# Autodesk Inventor assembly: Leg_joint_roll_pitch
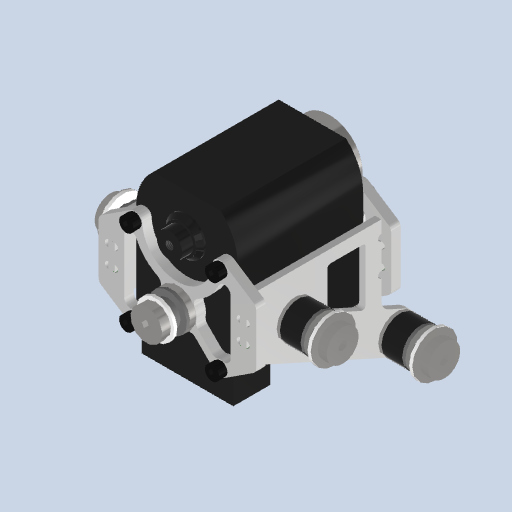
[picture p0: Inventor's stored thumbnail of the model, 512x512]
Saved by Autodesk Inventor 2022 (Build 260153000, 153)
## iProperties
Created: 2022-06-15
Part Number: Leg_joint_roll_pitch
Document SubType Name: Assembly
Designer: Masato Kubotera
Author: Masato Kubotera
## Documents named in this file (21)
- C:\Users\MasatoKubotera\Desktop\SUSTAINA-OP\LowerBody\Leg_joint\Leg_joint_roll_pitch.iam
- C:\Users\MasatoKubotera\Desktop\SUSTAINA-OP\LowerBody\Leg_joint\Leg_joint_pitch_frame.ipt
- C:\Users\MasatoKubotera\Desktop\SUSTAINA-OP\LowerBody\Leg_joint\Leg_joint_roll_frame.ipt
- C:\Users\MasatoKubotera\Desktop\SUSTAINA-OP\ReadyMade\KONDO\B3M-SC-1170-A_with_ClampHorn.iam
- C:\Users\MasatoKubotera\Desktop\SUSTAINA-OP\ReadyMade\InsertNut\S4-05-3W.ipt
- C:\Users\MasatoKubotera\Desktop\SUSTAINA-OP\ReadyMade\InsertNut\SF419.ipt
- C:\Users\MasatoKubotera\Desktop\SUSTAINA-OP\ReadyMade\Spacer\SLSBF6-39.5-M4-N4.ipt
- C:\Users\MasatoKubotera\Desktop\SUSTAINA-OP\ReadyMade\Washer\UUW-0412-10H.ipt
- C:\Users\MasatoKubotera\Desktop\SUSTAINA-OP\ReadyMade\Washer\CCC-0612-65B.ipt
- C:\Users\MasatoKubotera\Desktop\SUSTAINA-OP\ReadyMade\Bush\80F-0603.ipt
- C:\Users\MasatoKubotera\Desktop\SUSTAINA-OP\ReadyMade\Screw\DBTS4-11-6-DHC.ipt
- C:\Users\MasatoKubotera\Desktop\SUSTAINA-OP\ReadyMade\Screw\DBTS4-11-8-DHC.ipt
- C:\Users\MasatoKubotera\Desktop\SUSTAINA-OP\ReadyMade\Screw\DBTS4-5-5-DHC.ipt
- C:\Users\MasatoKubotera\Desktop\SUSTAINA-OP\ReadyMade\Screw\DBTS4-10-4-DHC.ipt
- C:\Users\MasatoKubotera\Desktop\SUSTAINA-OP\ReadyMade\Washer\UUW-0412-20H.ipt
- C:\Users\MasatoKubotera\Desktop\SUSTAINA-OP\ReadyMade\Washer\CC-0612-50B.ipt
- C:\Users\MasatoKubotera\Desktop\SUSTAINA-OP\ReadyMade\Washer\TT-0612-10.ipt
- C:\Users\MasatoKubotera\Desktop\SUSTAINA-OP\ReadyMade\Washer\TT-0814-10.ipt
- C:\Users\MasatoKubotera\Desktop\SUSTAINA-OP\ReadyMade\Washer\UUW-0614-03H.ipt
- C:\Users\MasatoKubotera\Desktop\SUSTAINA-OP\ReadyMade\Screw\FC-2620EB.ipt
- C:\Users\MasatoKubotera\Desktop\SUSTAINA-OP\ReadyMade\Screw\FC-2615EB.ipt
## Components (49 placed, 20 different names)
1. Leg_joint_pitch_frame:1 — 挿入:1, メイト:3, メイト:4, フラッシュ:2, フラッシュ:3, 挿入:13, 挿入:15, 挿入:16
2. Leg_joint_roll_frame:1 — 挿入:3, 角度:1, 挿入:5, 挿入:6, 挿入:7, 挿入:8, メイト:3, メイト:4, フラッシュ:2, メイト:5, メイト:6, 挿入:31, 挿入:48, 挿入:49, 挿入:50, 挿入:51
3. Leg_joint_pitch_frame:2 — 挿入:2, メイト:5, メイト:6, フラッシュ:3, 挿入:14, 挿入:17, 挿入:18
4. Leg_joint_roll_frame:2 — 挿入:4, 角度:2, 挿入:9, 挿入:10, 挿入:11, 挿入:12, 挿入:32, 挿入:52, 挿入:53
5. SLSBF6-39.5-M4-N4:1 — 挿入:13, 挿入:14
6. UUW-0412-10H:1 — 挿入:15, 挿入:19, 挿入:27
7. UUW-0412-10H:2 — 挿入:16, 挿入:20, 挿入:29
8. UUW-0412-10H:3 — 挿入:17, 挿入:21, 挿入:28
9. UUW-0412-10H:4 — 挿入:18, 挿入:22, 挿入:30
10. CCC-0612-65B:1 — 挿入:19, 挿入:23
11. CCC-0612-65B:2 — 挿入:20, 挿入:24
12. CCC-0612-65B:3 — 挿入:21, 挿入:25
13. CCC-0612-65B:4 — 挿入:22, 挿入:26
14. 80F-0603:1 — 挿入:23
15. 80F-0603:2 — 挿入:24
16. 80F-0603:3 — 挿入:25
17. 80F-0603:4 — 挿入:26
18. B3M-SC-1170-A_with_ClampHorn:1 [sub-assembly] — メイト:1, メイト:2, フラッシュ:1, 挿入:5, 挿入:6, 挿入:7, 挿入:8, 挿入:9, 挿入:10, 挿入:11, 挿入:12
19. S4-05-3W:1 — 挿入:3, 角度:1
20. SF419:1 — 挿入:1
21. S4-05-3W:2 — 挿入:4, 角度:2
22. SF419:2 — 挿入:2
23. UUW-0412-10H:5 — 挿入:32, 挿入:33, 挿入:37
24. UUW-0412-20H:1 — 挿入:31, 挿入:34, 挿入:36
25. CC-0612-50B:1 — 挿入:33, 挿入:35
26. 80F-0603:5 — 挿入:34
27. 80F-0603:6 — 挿入:35
28. TT-0612-10:1 — 挿入:38
29. TT-0612-10:2 — 挿入:39
30. TT-0814-10:1 — 挿入:42
31. UUW-0614-03H:1 — 挿入:40, 挿入:42
32. TT-0814-10:2 — 挿入:43
33. UUW-0614-03H:2 — 挿入:41, 挿入:43
34. TT-0814-10:3 — 挿入:46
35. UUW-0614-03H:3 — 挿入:44, 挿入:46
36. TT-0814-10:4 — 挿入:47
37. UUW-0614-03H:4 — 挿入:45, 挿入:47
38. FC-2620EB:1 — 挿入:48
39. FC-2620EB:2 — 挿入:49
40. FC-2620EB:3 — 挿入:50
41. FC-2620EB:4 — 挿入:51
42. FC-2615EB:1 — 挿入:52
43. FC-2615EB:2 — 挿入:53
44. DBTS4-11-6-DHC:1 — 挿入:27, 挿入:40
45. DBTS4-11-6-DHC:2 — 挿入:28, 挿入:41
46. DBTS4-11-8-DHC:1 — 挿入:29, 挿入:44
47. DBTS4-11-8-DHC:2 — 挿入:30, 挿入:45
48. DBTS4-5-5-DHC:1 — 挿入:36, 挿入:38
49. DBTS4-10-4-DHC:1 — 挿入:37, 挿入:39
## Relationships (64: Insert 53, Mate 6, Flush 3, Angle 2)
- メイト:1 [Mate]: B3M-SC-1170-A_with_ClampHorn:1
- メイト:2 [Mate]: B3M-SC-1170-A_with_ClampHorn:1
- フラッシュ:1 [Flush]: B3M-SC-1170-A_with_ClampHorn:1
- 挿入:1 [Insert]: Leg_joint_pitch_frame:1 ↔ SF419:1
- 挿入:2 [Insert]: Leg_joint_pitch_frame:2 ↔ SF419:2
- 挿入:3 [Insert]: Leg_joint_roll_frame:1 ↔ S4-05-3W:1
- 挿入:4 [Insert]: Leg_joint_roll_frame:2 ↔ S4-05-3W:2
- 角度:1 [Angle] (0 deg): Leg_joint_roll_frame:1 ↔ S4-05-3W:1
- 角度:2 [Angle] (0 deg): Leg_joint_roll_frame:2 ↔ S4-05-3W:2
- 挿入:5 [Insert]: Leg_joint_roll_frame:1 ↔ B3M-SC-1170-A_with_ClampHorn:1
- 挿入:6 [Insert]: Leg_joint_roll_frame:1 ↔ B3M-SC-1170-A_with_ClampHorn:1
- 挿入:7 [Insert]: Leg_joint_roll_frame:1 ↔ B3M-SC-1170-A_with_ClampHorn:1
- 挿入:8 [Insert]: Leg_joint_roll_frame:1 ↔ B3M-SC-1170-A_with_ClampHorn:1
- 挿入:9 [Insert]: Leg_joint_roll_frame:2 ↔ B3M-SC-1170-A_with_ClampHorn:1
- 挿入:10 [Insert]: Leg_joint_roll_frame:2 ↔ B3M-SC-1170-A_with_ClampHorn:1
- 挿入:11 [Insert]: Leg_joint_roll_frame:2 ↔ B3M-SC-1170-A_with_ClampHorn:1
- 挿入:12 [Insert]: Leg_joint_roll_frame:2 ↔ B3M-SC-1170-A_with_ClampHorn:1
- メイト:3 [Mate] (0.025 mm): Leg_joint_pitch_frame:1 ↔ Leg_joint_roll_frame:1
- メイト:4 [Mate] (0.025 mm): Leg_joint_pitch_frame:1 ↔ Leg_joint_roll_frame:1
- フラッシュ:2 [Flush]: Leg_joint_pitch_frame:1 ↔ Leg_joint_roll_frame:1
- メイト:5 [Mate] (0.025 mm): Leg_joint_roll_frame:1 ↔ Leg_joint_pitch_frame:2
- メイト:6 [Mate] (0.025 mm): Leg_joint_roll_frame:1 ↔ Leg_joint_pitch_frame:2
- フラッシュ:3 [Flush]: Leg_joint_pitch_frame:1 ↔ Leg_joint_pitch_frame:2
- 挿入:13 [Insert]: Leg_joint_pitch_frame:1 ↔ SLSBF6-39.5-M4-N4:1
- 挿入:14 [Insert]: Leg_joint_pitch_frame:2 ↔ SLSBF6-39.5-M4-N4:1
- 挿入:15 [Insert]: Leg_joint_pitch_frame:1 ↔ UUW-0412-10H:1
- 挿入:16 [Insert]: Leg_joint_pitch_frame:1 ↔ UUW-0412-10H:2
- 挿入:17 [Insert]: Leg_joint_pitch_frame:2 ↔ UUW-0412-10H:3
- 挿入:18 [Insert]: Leg_joint_pitch_frame:2 ↔ UUW-0412-10H:4
- 挿入:19 [Insert]: UUW-0412-10H:1 ↔ CCC-0612-65B:1
- 挿入:20 [Insert]: UUW-0412-10H:2 ↔ CCC-0612-65B:2
- 挿入:21 [Insert]: UUW-0412-10H:3 ↔ CCC-0612-65B:3
- 挿入:22 [Insert]: UUW-0412-10H:4 ↔ CCC-0612-65B:4
- 挿入:23 [Insert]: CCC-0612-65B:1 ↔ 80F-0603:1
- 挿入:24 [Insert]: CCC-0612-65B:2 ↔ 80F-0603:2
- 挿入:25 [Insert]: CCC-0612-65B:3 ↔ 80F-0603:3
- 挿入:26 [Insert]: CCC-0612-65B:4 ↔ 80F-0603:4
- 挿入:27 [Insert]: UUW-0412-10H:1 ↔ DBTS4-11-6-DHC:1
- 挿入:28 [Insert]: UUW-0412-10H:3 ↔ DBTS4-11-6-DHC:2
- 挿入:29 [Insert]: UUW-0412-10H:2 ↔ DBTS4-11-8-DHC:1
- 挿入:30 [Insert]: UUW-0412-10H:4 ↔ DBTS4-11-8-DHC:2
- 挿入:31 [Insert]: Leg_joint_roll_frame:1 ↔ UUW-0412-20H:1
- 挿入:32 [Insert]: Leg_joint_roll_frame:2 ↔ UUW-0412-10H:5
- 挿入:33 [Insert]: UUW-0412-10H:5 ↔ CC-0612-50B:1
- 挿入:34 [Insert]: UUW-0412-20H:1 ↔ 80F-0603:5
- 挿入:35 [Insert]: CC-0612-50B:1 ↔ 80F-0603:6
- 挿入:36 [Insert]: UUW-0412-20H:1 ↔ DBTS4-5-5-DHC:1
- 挿入:37 [Insert]: UUW-0412-10H:5 ↔ DBTS4-10-4-DHC:1
- 挿入:38 [Insert]: TT-0612-10:1 ↔ DBTS4-5-5-DHC:1
- 挿入:39 [Insert]: TT-0612-10:2 ↔ DBTS4-10-4-DHC:1
- 挿入:40 [Insert]: UUW-0614-03H:1 ↔ DBTS4-11-6-DHC:1
- 挿入:41 [Insert]: UUW-0614-03H:2 ↔ DBTS4-11-6-DHC:2
- 挿入:42 [Insert]: TT-0814-10:1 ↔ UUW-0614-03H:1
- 挿入:43 [Insert]: TT-0814-10:2 ↔ UUW-0614-03H:2
- 挿入:44 [Insert]: UUW-0614-03H:3 ↔ DBTS4-11-8-DHC:1
- 挿入:45 [Insert]: UUW-0614-03H:4 ↔ DBTS4-11-8-DHC:2
- 挿入:46 [Insert]: TT-0814-10:3 ↔ UUW-0614-03H:3
- 挿入:47 [Insert]: TT-0814-10:4 ↔ UUW-0614-03H:4
- 挿入:48 [Insert]: Leg_joint_roll_frame:1 ↔ FC-2620EB:1
- 挿入:49 [Insert]: Leg_joint_roll_frame:1 ↔ FC-2620EB:2
- 挿入:50 [Insert]: Leg_joint_roll_frame:1 ↔ FC-2620EB:3
- 挿入:51 [Insert]: Leg_joint_roll_frame:1 ↔ FC-2620EB:4
- 挿入:52 [Insert]: Leg_joint_roll_frame:2 ↔ FC-2615EB:1
- 挿入:53 [Insert]: Leg_joint_roll_frame:2 ↔ FC-2615EB:2
